# Autodesk Inventor assembly: Rear_Train
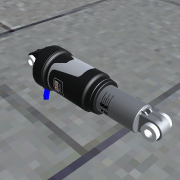
[picture p0: Inventor's stored thumbnail of the model, 180x180]
Saved by Autodesk Inventor 2014 (Build 180170000, 170)
## iProperties
Created: 2015-04-04
Part Number: Rear_Train
Document SubType Name: Assembly
Designer: Yann
Author: Yann
## Documents named in this file (2)
- C:\Users\Yann\Documents\GitHub\BIKAIR_CAD\Source\Rear_Train\Rear_Train.iam
- C:\Users\Yann\Documents\GitHub\BIKAIR_CAD\Source\Rear_Train\Suspension\Rock Shox\Rock Shox.iam
## Components (1 placed, 1 different names)
1. Rock Shox:1 [sub-assembly] — Placage:1
## Relationships (1: Mate 1)
- Placage:1 [Mate]: Rock Shox:1
